# Autodesk Inventor assembly: endAssembly
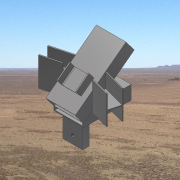
[picture p0: Inventor's stored thumbnail of the model, 180x180]
Saved by Autodesk Inventor 2014 SP1 (Build 180222100, 222)
## iProperties
Created: 2013-12-03
Part Number: endAssembly
Document SubType Name: Assembly
Designer: Dave
Author: Dave
## Documents named in this file (5)
- C:\Users\Dave\Desktop\hera-cad\support\endAssembly.iam
- C:\Users\Dave\Desktop\hera-cad\support\endHoriz.ipt
- C:\Users\Dave\Desktop\hera-cad\support\end37.ipt
- C:\Users\Dave\Desktop\hera-cad\support\endVert1.ipt
- C:\Users\Dave\Desktop\hera-cad\support\end37channel.ipt
## Components (5 placed, 4 different names)
1. endHoriz:1 — Mate:1, Flush:3
2. end37:1 — Mate:1, Mate:5, Flush:3, Flush:4, Flush:5, Mate:7, Mate:8
3. endVert1:1 — Mate:7
4. end37channel:1 — Mate:5, Flush:4, Flush:5
5. endVert1:2 — Mate:8
## Relationships (7: Mate 4, Flush 3)
- Mate:1: endHoriz:1 ↔ end37:1
- Mate:5: end37:1 ↔ end37channel:1
- Flush:3: endHoriz:1 ↔ end37:1
- Flush:4 (44.45 mm): end37:1 ↔ end37channel:1
- Flush:5 (-16.51 mm): end37:1 ↔ end37channel:1
- Mate:7: end37:1 ↔ endVert1:1
- Mate:8: end37:1 ↔ endVert1:2
